# Autodesk Inventor assembly: batteriesfourpack
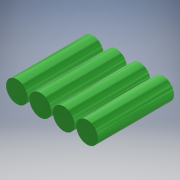
[picture p0: Inventor's stored thumbnail of the model, 180x180]
Saved by Autodesk Inventor 2022.3 (Build 263350000, 350)
## iProperties
Created: 2021-10-06
Part Number: batteriesfourpack
Document SubType Name: Assembly
Designer: Bowen O'Steen
Author: Bowen O'Steen
## Documents named in this file (2)
- C:\Users\gwhen\OneDrive\Desktop\Vault\Designs\MEMESat\MemeSat\Engineering Data\MemeSat\Subsystems\BoBa\batteriesfourpack.iam
- C:\Users\gwhen\OneDrive\Desktop\Vault\Designs\MEMESat\MemeSat\Engineering Data\MemeSat\Subsystems\BoBa\batterysingle.ipt
## Components (4 placed, 1 different names)
1. batterysingle:1 — Mate:1, Mate:2, Flush:1
2. batterysingle:2
3. batterysingle:3
4. batterysingle:4
## Component patterns: (4 elements, first: batterysingle:1)
## Relationships (3: Mate 2, Flush 1)
- Mate:1: batterysingle:1
- Mate:2: batterysingle:1
- Flush:1: batterysingle:1
